# Autodesk Inventor assembly: skrzydlo_ster_MIR
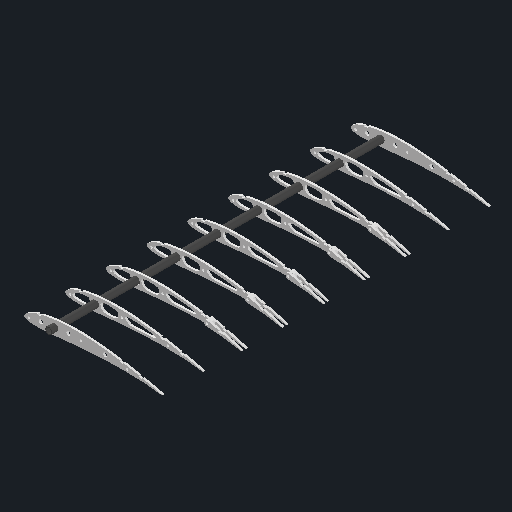
[picture p0: Inventor's stored thumbnail of the model, 512x512]
Saved by Autodesk Inventor 2023 (Build 270158000, 158)
## iProperties
Created: 2023-01-05
Part Number: skrzydlo_ster_MIR
Document SubType Name: Assembly
Designer: szykr
Author: szykr
## Documents named in this file (5)
- D:\Folder Instalacyjny\GitHub Pliki\Solaris\new model\Skrzydlo_ster_mir\skrzydlo_ster_MIR.iam
- D:\Folder Instalacyjny\GitHub Pliki\Solaris\new model\Skrzydlo_ster_mir\Wingspar trochemniejnizpol metrowy_MIR.ipt
- D:\Folder Instalacyjny\GitHub Pliki\Solaris\new model\Skrzydlo_ster_mir\Żerbo montaż_MIR.ipt
- D:\Folder Instalacyjny\GitHub Pliki\Solaris\new model\Skrzydlo_ster_mir\Zebro_lotka_MIR.iam
- D:\Folder Instalacyjny\GitHub Pliki\Solaris\new model\Skrzydlo_ster_mir\Żebro default_MIR.ipt
## Components (10 placed, 4 different names)
1. Wingspar trochemniejnizpol metrowy_MIR:1
2. Żerbo montaż_MIR:1
3. Żerbo montaż_MIR:2
4. Żebro default_MIR:2
5. Żebro default_MIR:1
6. Zebro_lotka_MIR:1 [sub-assembly]
7. Zebro_lotka_MIR:2 [sub-assembly]
8. Zebro_lotka_MIR:3 [sub-assembly]
9. Zebro_lotka_MIR:4 [sub-assembly]
10. Zebro_lotka_MIR:5 [sub-assembly]
## Component patterns: (1 elements, first: Żebro default_MIR:2), (1 elements, first: Żebro default_MIR:1), (5 elements, first: Zebro_lotka_MIR:1)
## Named parameters: dlugosc = 472.43 mm, pre_zebra = 1, post_zebra = 1, lotki = 5, ilosc_zeber = 8, spacing = 59.054 mm
